# Autodesk Inventor assembly: AssembledProduct
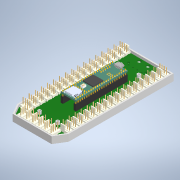
[picture p0: Inventor's stored thumbnail of the model, 180x180]
Saved by Autodesk Inventor 2022 (Build 260153000, 153)
## iProperties
Created: 2021-05-25
Part Number: AssembledProduct
Document SubType Name: Assembly
Designer: Collin
Author: Collin
## Documents named in this file (4)
- H:\Projects\RGB Controller\Teensy-PC_RGB_Controller\2 PCB\CAD\V3\AssembledProduct.iam
- H:\Projects\RGB Controller\Teensy-PC_RGB_Controller\2 PCB\CAD\CaseBottomV2.ipt
- H:\Projects\RGB Controller\Teensy-PC_RGB_Controller\2 PCB\CAD\V3\CircuitBoardV2.iam
- H:\Projects\RGB Controller\Teensy-PC_RGB_Controller\2 PCB\CAD\teensy-4-1-development-board-1.snapshot.5\Teensy 4.1 (With Headers).iam
## Components (3 placed, 3 different names)
1. CaseBottomV2:1 — Mate:2, Mate:3, Mate:4
2. CircuitBoardV2:1 [sub-assembly] — Mate:2, Mate:3, Mate:4, Mate:5, Mate:6, Mate:7
3. Teensy 4.1 (With Headers):1 [sub-assembly] — Mate:5, Mate:6, Mate:7
## Relationships (6: Mate 6)
- Mate:2: CaseBottomV2:1 ↔ CircuitBoardV2:1
- Mate:3: CaseBottomV2:1 ↔ CircuitBoardV2:1
- Mate:4: CaseBottomV2:1 ↔ CircuitBoardV2:1
- Mate:5: CircuitBoardV2:1 ↔ Teensy 4.1 (With Headers):1
- Mate:6: CircuitBoardV2:1 ↔ Teensy 4.1 (With Headers):1
- Mate:7: CircuitBoardV2:1 ↔ Teensy 4.1 (With Headers):1
